# Autodesk Inventor assembly: MAIN
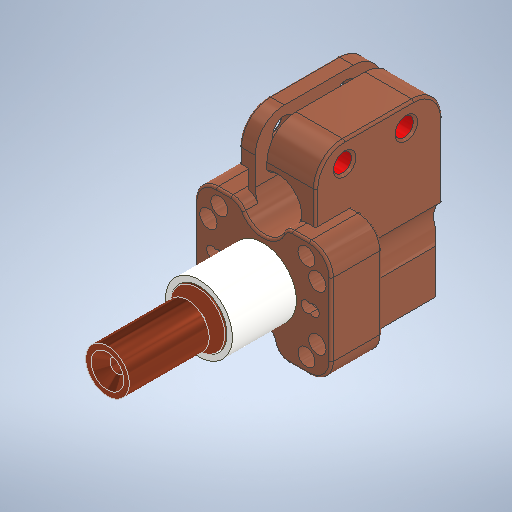
[picture p0: Inventor's stored thumbnail of the model, 512x512]
Saved by Autodesk Inventor 2025.2 (Build 292293000, 293)
## iProperties
Created: 2025-08-19
Part Number: MAIN
Document SubType Name: Assembly
Designer: wangg
Author: wangg
## Documents named in this file (4)
- C:\Users\wangg\OneDrive\桌面\Crazy_Dragon_LC\MAIN.iam
- C:\Users\wangg\OneDrive\桌面\Crazy_Dragon_LC\Purchased Parts\NF-Crazy Volcano heat block\NF-Crazy Volcano heat block\NF-Crazy Volcano heat block.ipt
- C:\Users\wangg\OneDrive\桌面\Crazy_Dragon_LC\Purchased Parts\Creality Spider Pro\Creality Spider Pro\Creality Spider Pro.ipt
- C:\Users\wangg\OneDrive\桌面\Crazy_Dragon_LC\Heatsink_HOTEND_WC_CHANNEL.ipt
## Components (3 placed, 3 different names)
1. NF-Crazy Volcano heat block:1 — Mate:1, Mate:2
2. Creality Spider Pro:1 — Mate:1, Mate:2
3. Heatsink_HOTEND_WC_CHANNEL:1
## Relationships (2: Mate 2)
- Mate:1: NF-Crazy Volcano heat block:1 ↔ Creality Spider Pro:1
- Mate:2: NF-Crazy Volcano heat block:1 ↔ Creality Spider Pro:1
